# Autodesk Inventor assembly: !gearbox
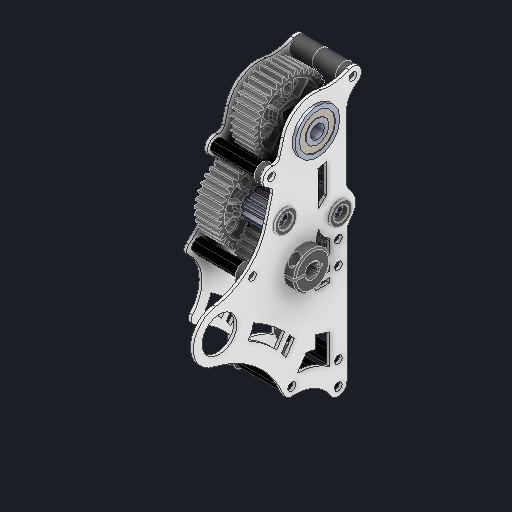
[picture p0: Inventor's stored thumbnail of the model, 512x512]
Saved by Autodesk Inventor 2024 (Build 280153000, 153)
## iProperties
Created: 2023-11-21
Part Number: !gearbox
Document SubType Name: Assembly
Designer: avere
Author: avere
## Documents named in this file (16)
- C:\Users\avere\Documents\rbp_cad\zoomba_v0.1\arm\gearbox.iam
- gearbox.iam
- C:\Users\avere\Documents\rbp_cad\zoomba_v0.1\chassis\custom_parts\reservoir_mount.ipt
- C:\Users\avere\Documents\rbp_cad\VEX-CAD-Inventor-1.41\Motion\Shaft HS\HS Bushing 0.1250.ipt
- C:\Users\avere\Documents\rbp_cad\VEX-CAD-Inventor-1.41\Motion\Gears\HS Gear\HS 12T Gear, No Insert.iam
- C:\Users\avere\Documents\rbp_cad\VEX-CAD-Inventor-1.41\Motion\Gears\HS Gear.iam
- C:\Users\avere\Documents\rbp_cad\VEX-CAD-Inventor-1.41\Motion\Gears\HS Gear\HS 36T Gear, No Insert.iam
- C:\Users\avere\Documents\rbp_cad\VEX-CAD-Inventor-1.41\Motion\Reference Files\Ball Bearing.ipt
- C:\Users\avere\Documents\rbp_cad\VEX-CAD-Inventor-1.41\Structure\Standoff\Standoff 1.00.ipt
- C:\Users\avere\Documents\rbp_cad\VEX-CAD-Inventor-1.41\Structure\Standoff.ipt
- C:\Users\avere\Documents\rbp_cad\VEX-CAD-Inventor-1.41\Motion\Spacers\Spacer Nylon .375 OD\NSpacer .375 OD x .125.ipt
- C:\Users\avere\Documents\rbp_cad\VEX-CAD-Inventor-1.41\Motion\Spacers\Spacer Nylon .375 OD.ipt
- C:\Users\avere\Documents\rbp_cad\VEX-CAD-Inventor-1.41\Motion\Shaft HS\Low Profile HS Shaft Collar.ipt
- C:\Users\avere\Documents\rbp_cad\VEX-CAD-Inventor-1.41\Motion\Shaft HS\HS Shaft Collar.ipt
- C:\Users\avere\Documents\rbp_cad\zoomba_v0.1\chassis\custom_parts\reservoir_mount_inner.ipt
- C:\Users\avere\Documents\rbp_cad\VEX-CAD-Inventor-1.41\Motion\Spacers\Spacer Nylon .375 OD\NSpacer .375 OD x .500.ipt
## Components (28 placed, 11 different names)
1. reservoir_mount:1 — Mate:1
2. HS Bushing 0.1250:1
3. HS Bushing 0.1250:2
4. HS Bushing 0.1250:3
5. HS 12T Gear, No Insert:1 [sub-assembly]
6. HS 12T Gear, No Insert:2 [sub-assembly]
7. HS 36T Gear, No Insert:3 [sub-assembly]
8. HS 36T Gear, No Insert:4 [sub-assembly]
9. HS 12T Gear, No Insert:5 [sub-assembly]
10. Ball Bearing:1
11. Standoff 1.00:1
12. NSpacer .375 OD x .125:1
13. NSpacer .375 OD x .125:2 — Insert:23
14. Standoff 1.00:3
15. NSpacer .375 OD x .125:3
16. HS 36T Gear, No Insert:6 [sub-assembly] — Insert:21
17. Low Profile HS Shaft Collar:1
18. HS Shaft Collar:1
19. reservoir_mount_inner:1 — Mate:1, Insert:20, Insert:25, Insert:27, Insert:29
20. Ball Bearing:2 — Insert:20, Insert:21
21. NSpacer .375 OD x .500:4 — Insert:22
22. NSpacer .375 OD x .500:5 — Insert:22, Insert:23
23. Standoff 1.00:4
24. NSpacer .375 OD x .125:6 — Insert:25
25. Standoff 1.00:5
26. NSpacer .375 OD x .125:7 — Insert:27
27. Standoff 1.00:6
28. NSpacer .375 OD x .125:8 — Insert:29
## Relationships (26: Insert 25, Mate 1)
- [Insert]: reservoir_mount:1 ↔ HS Bushing 0.1250:2
- [Insert]: reservoir_mount:1 ↔ HS Bushing 0.1250:3
- [Insert]: reservoir_mount:1 ↔ HS Bushing 0.1250:1
- [Insert] (1.5875 mm): HS Bushing 0.1250:1 ↔ HS 12T Gear, No Insert:1
- [Insert] (1.5875 mm): HS Bushing 0.1250:2 ↔ HS 36T Gear, No Insert:3
- [Insert]: HS 12T Gear, No Insert:2 ↔ HS 36T Gear, No Insert:3
- [Insert] (14.2875 mm): HS Bushing 0.1250:3 ↔ HS 36T Gear, No Insert:4
- [Insert]: HS 36T Gear, No Insert:4 ↔ HS 12T Gear, No Insert:5
- [Insert]: Standoff 1.00:1 ↔ NSpacer .375 OD x .125:1
- [Insert]: reservoir_mount:1 ↔ NSpacer .375 OD x .125:1
- [Insert]: reservoir_mount:1 ↔ NSpacer .375 OD x .125:2
- [Insert]: Standoff 1.00:3 ↔ NSpacer .375 OD x .125:3
- [Insert]: reservoir_mount:1 ↔ NSpacer .375 OD x .125:3
- [Insert]: reservoir_mount:1 ↔ Ball Bearing:1
- [Insert]: HS Bushing 0.1250:2 ↔ Low Profile HS Shaft Collar:1
- Mate:1: reservoir_mount:1 ↔ reservoir_mount_inner:1
- Insert:20: reservoir_mount_inner:1 ↔ Ball Bearing:2
- Insert:21: HS 36T Gear, No Insert:6 ↔ Ball Bearing:2
- Insert:22: NSpacer .375 OD x .500:4 ↔ NSpacer .375 OD x .500:5
- Insert:23: NSpacer .375 OD x .125:2 ↔ NSpacer .375 OD x .500:5
- [Insert]: Standoff 1.00:4 ↔ NSpacer .375 OD x .125:6
- Insert:25: reservoir_mount_inner:1 ↔ NSpacer .375 OD x .125:6
- [Insert]: Standoff 1.00:5 ↔ NSpacer .375 OD x .125:7
- Insert:27: reservoir_mount_inner:1 ↔ NSpacer .375 OD x .125:7
- [Insert]: Standoff 1.00:6 ↔ NSpacer .375 OD x .125:8
- Insert:29: reservoir_mount_inner:1 ↔ NSpacer .375 OD x .125:8
## Named parameters: d418_d414 = 0 mm, d26_d418_d414 = 0 mm, d28_d26_d418_d414 = 0 mm, d30_d28_d26_d418_d414 = 0 mm
